# Autodesk Inventor assembly: Assembly
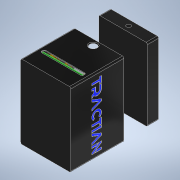
[picture p0: Inventor's stored thumbnail of the model, 180x180]
Saved by Autodesk Inventor 2021 (Build 250183000, 183)
## iProperties
Created: 2023-01-24
Part Number: Assembly
Document SubType Name: Assembly
Designer: nicho
Author: nicho
## Documents named in this file (5)
- C:\Users\nicho\Documents\Work\Tractian\TRACTIAN-Challenge\Mechanics\Assembly.iam
- C:\Users\nicho\Documents\Work\Tractian\TRACTIAN-Challenge\Mechanics\PCB.ipt
- C:\Users\nicho\Documents\Work\Tractian\TRACTIAN-Challenge\Mechanics\Case - Base.ipt
- C:\Users\nicho\Documents\Work\Tractian\TRACTIAN-Challenge\Mechanics\Battery.ipt
- C:\Users\nicho\Documents\Work\Tractian\TRACTIAN-Challenge\Mechanics\Case - Tampa.ipt
## Components (4 placed, 4 different names)
1. PCB:1 — Coincidente:1, Coincidente:2, Coincidente:3
2. Case - Base:1 — Coincidente:1, Coincidente:2, Coincidente:3, Coincidente:4, Coincidente:5, Coincidente:6, Coincidente:7, Conjunto de gaveta:1, Coincidente:8
3. Battery:1 — Coincidente:4, Coincidente:5, Coincidente:8
4. Case - Tampa:1 — Coincidente:6, Coincidente:7, Conjunto de gaveta:1
## Relationships (9: Mate 8, TranslationJoint 1)
- Coincidente:1 [Mate]: PCB:1 ↔ Case - Base:1
- Coincidente:2 [Mate]: PCB:1 ↔ Case - Base:1
- Coincidente:3 [Mate]: PCB:1 ↔ Case - Base:1
- Coincidente:4 [Mate]: Case - Base:1 ↔ Battery:1
- Coincidente:5 [Mate]: Case - Base:1 ↔ Battery:1
- Coincidente:6 [Mate]: Case - Base:1 ↔ Case - Tampa:1
- Coincidente:7 [Mate]: Case - Base:1 ↔ Case - Tampa:1
- Conjunto de gaveta:1 [TranslationJoint]: Case - Base:1 ↔ Case - Tampa:1
- Coincidente:8 [Mate] (5.5 mm): Case - Base:1 ↔ Battery:1
